# Autodesk Inventor assembly: dog_driver_5.brd
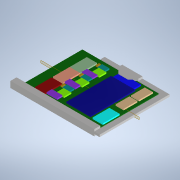
[picture p0: Inventor's stored thumbnail of the model, 180x180]
Saved by Autodesk Inventor 2020 (Build 240168000, 168)
## iProperties
Created: 2019-08-29
Part Number: dog_driver_5.brd
Document SubType Name: Assembly
Designer: psrob
Author: psrob
## Documents named in this file (21)
- E:\projects-2\project dog gen2\hardware\ele_3d_3\dog_driver_5.brd.iam
- E:\projects-2\project dog gen2\hardware\ele_3d_3\dog_driver_5.brd_Outline.ipt
- E:\projects-2\project dog gen2\hardware\ele_3d_3\ARDUINO_PRO_MINI, ARDUINO1_ARDUINO_PRO_MINI_1.ipt
- E:\projects-2\project dog gen2\hardware\ele_3d_3\EIA3528, 47UF_3.ipt
- E:\projects-2\project dog gen2\hardware\ele_3d_3\0402, 0_1UF_5.ipt
- E:\projects-2\project dog gen2\hardware\ele_3d_3\0603, 10UF_11.ipt
- E:\projects-2\project dog gen2\hardware\ele_3d_3\0805, 0_33_F_13.ipt
- E:\projects-2\project dog gen2\hardware\ele_3d_3\0603, 0_1UF_15.ipt
- E:\projects-2\project dog gen2\hardware\ele_3d_3\53261-04, 53261-04_17.ipt
- E:\projects-2\project dog gen2\hardware\ele_3d_3\TO252, 7805DT_22.ipt
- E:\projects-2\project dog gen2\hardware\ele_3d_3\SCREWTERMINAL-5MM-2, J1_SCREWTERMINAL-5MM-2_24.ipt
- E:\projects-2\project dog gen2\hardware\ele_3d_3\SCREWTERMINAL-5MM-2, J2_SCREWTERMINAL-5MM-2_26.ipt
- E:\projects-2\project dog gen2\hardware\ele_3d_3\SCREWTERMINAL-5MM-2, J3_SCREWTERMINAL-5MM-2_28.ipt
- E:\projects-2\project dog gen2\hardware\ele_3d_3\SCREWTERMINAL-5MM-2, J4_SCREWTERMINAL-5MM-2_30.ipt
- E:\projects-2\project dog gen2\hardware\ele_3d_3\6410-06, 22-27-2061-06_32.ipt
- E:\projects-2\project dog gen2\hardware\ele_3d_3\R2512, 0_22_34.ipt
- E:\projects-2\project dog gen2\hardware\ele_3d_3\0603, 10K_38.ipt
- E:\projects-2\project dog gen2\hardware\ele_3d_3\6410-04, 22-27-2041-04_43.ipt
- E:\projects-2\project dog gen2\hardware\ele_3d_3\SOP65P640X120-24N, TCA9548APWR_46.ipt
- E:\projects-2\project dog gen2\hardware\ele_3d_3\SOIC8TP, A4950ELJTR-T_48.ipt
- E:\projects-2\project dog gen2\hardware\ele_3d_3\pcb_holder_5.ipt
## Components (35 placed, 35 different names)
1. dog_driver_5.brd_Outline:1 — Flush:1
2. ARDUINO1_2
3. C1_4
4. C2_6
5. C3_7
6. C4_8
7. C5_9
8. C6_10
9. C7_12
10. C8_14
11. C9_16
12. E1_18
13. E2_19
14. E3_20
15. EA_21
16. IC1_23
17. J1_25
18. J2_27
19. J3_29
20. J4_31
21. J5_33
22. R1_35
23. R2_36
24. R3_37
25. R4_39
26. R5_40
27. R6_41
28. R7_42
29. SE_44
30. SW_45
31. U1_47
32. U2_49
33. U3_50
34. U4_51
35. pcb_holder_5:1 — Flush:1
## Relationships (1: Flush 1)
- Flush:1: dog_driver_5.brd_Outline:1 ↔ pcb_holder_5:1
